# Autodesk Inventor assembly: Assembly1
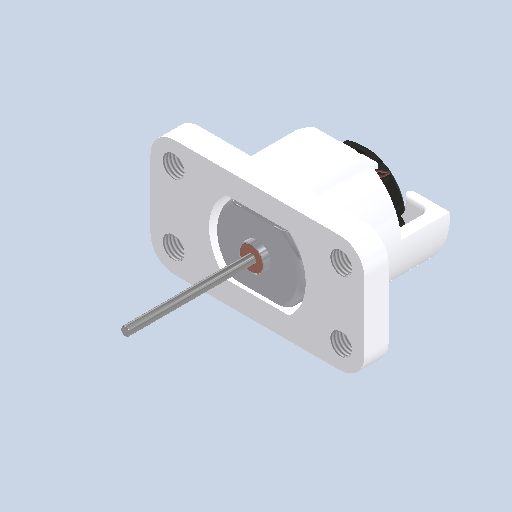
[picture p0: Inventor's stored thumbnail of the model, 512x512]
Saved by Autodesk Inventor 2025.3 (Build 293356000, 356)
## iProperties
Created: 2026-04-10
Part Number: Assembly1
Document SubType Name: Assembly
Designer: abdul
Author: abdul
## Documents named in this file (3)
- D:\BO\Assembly1.iam
- C:\Users\abdul\Downloads\dc motor.ipt
- D:\BO\dc motor mount-FINAL.ipt
## Components (2 placed, 2 different names)
1. dc motor:1 — Mate:1, Mate:2, Mate:3
2. dc motor mount-FINAL:1 — Mate:1, Mate:2, Mate:3
## Relationships (3: Mate 3)
- Mate:1: dc motor:1 ↔ dc motor mount-FINAL:1
- Mate:2: dc motor:1 ↔ dc motor mount-FINAL:1
- Mate:3: dc motor:1 ↔ dc motor mount-FINAL:1
